# Autodesk Inventor assembly: CopleyAccelus_full.ipt
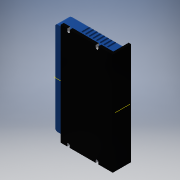
[picture p0: Inventor's stored thumbnail of the model, 180x180]
Saved by Autodesk Inventor 2019 (Build 230136000, 136)
## iProperties
Created: 2019-05-17
Part Number: CopleyAccelus_full.ipt
Document SubType Name: Assembly
Designer: Jorian Bruslind
Author: Jorian Bruslind
## Documents named in this file (4)
- E:\Downloads\Robot_Controller_Models\CopleyAccelus_full.ipt.iam
- E:\Downloads\Robot_Controller_Models\CopleyAccelus.ipt
- E:\Downloads\Robot_Controller_Models\DB15_F.ipt
- E:\Downloads\Robot_Controller_Models\DB25_F.ipt
## Components (3 placed, 3 different names)
1. CopleyAccelus:1 — Mate:1, Mate:2, Mate:3, Mate:4, Mate:5, Mate:6
2. DB15_F:1 — Mate:3, Mate:4, Mate:5
3. DB25_F:1 — Mate:1, Mate:2, Mate:6
## Relationships (6: Mate 6)
- Mate:1: CopleyAccelus:1 ↔ DB25_F:1
- Mate:2: CopleyAccelus:1 ↔ DB25_F:1
- Mate:3: CopleyAccelus:1 ↔ DB15_F:1
- Mate:4: CopleyAccelus:1 ↔ DB15_F:1
- Mate:5: CopleyAccelus:1 ↔ DB15_F:1
- Mate:6: CopleyAccelus:1 ↔ DB25_F:1
